# Autodesk Inventor assembly: four_square_base
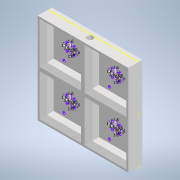
[picture p0: Inventor's stored thumbnail of the model, 180x180]
Saved by Autodesk Inventor 2021 (Build 250183000, 183)
## iProperties
Created: 2020-12-08
Part Number: four_square_base
Document SubType Name: Assembly
Designer: Luke Kamols
Author: Luke Kamols
## Documents named in this file (2)
- C:\Users\Luke Kamols\OneDrive\Documents\Other\Chess\four_square_base.iam
- C:\Users\Luke Kamols\OneDrive\Documents\Other\Chess\one-square.ipt
## Components (4 placed, 1 different names)
1. one-square:1 — Mate:1, Flush:1, Flush:2, Mate:2, Flush:3, Flush:4
2. one-square:2 — Mate:1, Flush:1, Flush:2, Flush:5, Mate:3
3. one-square:3 — Mate:2, Flush:3, Flush:4, Mate:4
4. one-square:4 — Flush:5, Mate:3, Mate:4
## Relationships (9: Flush 5, Mate 4)
- Mate:1: one-square:1 ↔ one-square:2
- Flush:1: one-square:1 ↔ one-square:2
- Flush:2: one-square:1 ↔ one-square:2
- Mate:2: one-square:1 ↔ one-square:3
- Flush:3: one-square:1 ↔ one-square:3
- Flush:4: one-square:1 ↔ one-square:3
- Flush:5: one-square:2 ↔ one-square:4
- Mate:3: one-square:2 ↔ one-square:4
- Mate:4: one-square:3 ↔ one-square:4
